# Autodesk Inventor assembly: Stator
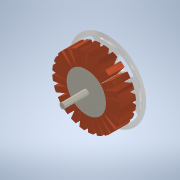
[picture p0: Inventor's stored thumbnail of the model, 180x180]
Saved by Autodesk Inventor 2020.2 (Build 242310000, 310)
## iProperties
Created: 2020-02-19
Part Number: Stator
Document SubType Name: Assembly
Designer: user
Author: user
## Documents named in this file (4)
- C:\Users\user\OneDrive\바탕 화면\CtrBox\Stator.iam
- C:\Users\user\OneDrive\바탕 화면\CtrBox\Stator Base.ipt
- C:\Users\user\OneDrive\바탕 화면\CtrBox\Stator Axis.ipt
- C:\Users\user\OneDrive\바탕 화면\CtrBox\Stator Coil.ipt
## Components (3 placed, 3 different names)
1. Stator Base:1 — Mate:1, Mate:2
2. Stator Axis:1 — Mate:1, Mate:2, Mate:3, Flush:1
3. Stator Coil:1 — Mate:3, Flush:1
## Relationships (4: Mate 3, Flush 1)
- Mate:1: Stator Base:1 ↔ Stator Axis:1
- Mate:2: Stator Base:1 ↔ Stator Axis:1
- Mate:3: Stator Axis:1 ↔ Stator Coil:1
- Flush:1: Stator Axis:1 ↔ Stator Coil:1
